# Autodesk Inventor assembly: Joint_0_1
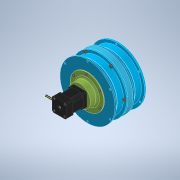
[picture p0: Inventor's stored thumbnail of the model, 180x180]
Saved by Autodesk Inventor 2021 (Build 250183000, 183)
## iProperties
Created: 2020-05-11
Part Number: Joint_0_1
Document SubType Name: Assembly
Designer: avi41
Mass: 3564.7 g
Surface Area: 4281.87 cm^2
Volume: 931.801 cm^3
Density: 3.8256 g/cm^3
Author: avi41
## Documents named in this file (15)
- C:\Users\avi41\Desktop\Robot Arm\CAD_files\Joint_0_1.iam
- C:\Users\avi41\Desktop\Robot Arm\CAD_files\DB41M024030-A.ipt
- C:\Users\avi41\Desktop\Robot Arm\CAD_files\PlanetaryGearbox_stage.iam
- C:\Users\avi41\Desktop\Robot Arm\CAD_files\Adapter_stages_planetary.ipt
- C:\Users\avi41\Documents\Inventor\Content Center Files\R2020\en-US\ANSI B18.3.4M(2)\ANSI B18.3.4M - M4 x 0.7 x 30(1).ipt
- C:\Users\avi41\Documents\Inventor\Content Center Files\R2020\en-US\ISO 4032(1)\ISO 4032 - M4DIN EN.ipt
- C:\Users\avi41\Desktop\Robot Arm\CAD_files\Adapter_motor_planetarygearbox.ipt
- C:\Users\avi41\Documents\Inventor\Content Center Files\R2020\en-US\ANSI B18.3.4M(2)\ANSI B18.3.4M - M3 x 0.5 x 8(1).ipt
- C:\Users\avi41\Documents\Inventor\Content Center Files\R2020\en-US\ISO 8738(1)\ISO 8738 - 3(1).ipt
- C:\Users\avi41\Documents\Inventor\Content Center Files\R2020\en-US\ISO 8738(1)\ISO 8738 - 4(1).ipt
- C:\Users\avi41\Desktop\Robot Arm\CAD_files\MB029-F_1.ipt
- C:\Users\avi41\Desktop\Robot Arm\CAD_files\MRA029BC010DSE00.iam
- C:\Users\avi41\Documents\Inventor\Content Center Files\R2021\en-US\ISO 7046-1 Z(2)\ISO 7046-1 - M2 x 12 - 4.8 - ZNF EN ISO.ipt
- C:\Users\avi41\Documents\Inventor\Content Center Files\R2021\en-US\ISO 4032(1)\ISO 4032 - M2DIN EN.ipt
- C:\Users\avi41\Documents\Inventor\Content Center Files\R2021\en-US\ISO 7046-1 Z(2)\ISO 7046-1 - M3 x 10 - 4.8 - ZNF EN ISO.ipt
## Components (55 placed, 14 different names)
1. PlanetaryGearbox_stage:1 [sub-assembly] — Mate:1, Mate:2, Flush:1, Mate:3, Mate:5, Mate:6, Mate:7, Mate:9, Mate:10, Mate:11, Mate:12, Mate:13, Mate:14, Mate:38, Mate:39, Mate:40, Mate:42, Mate:43, Mate:44, Mate:53, Mate:54, Mate:55, Mate:56
2. DB41M024030-A:1 — Mate:3, Mate:15, Mate:16, Mate:29
3. PlanetaryGearbox_stage:2 [sub-assembly] — Mate:5, Mate:6, Mate:8, Mate:11
4. Adapter_stages_planetary:1 — Mate:7, Mate:8, Mate:9, Mate:10
5. Adapter_motor_planetarygearbox:1 — Mate:12, Mate:13, Mate:14, Mate:15, Mate:16, Mate:29, Mate:58, Mate:59, Mate:60, Mate:61, Flush:2, Flush:3, Flush:4, Flush:5, Mate:62, Mate:63, Mate:64
6. MB029-F_1:1 — Mate:62, Mate:63, Mate:64
7. MRA029BC010DSE00:1 [sub-assembly] — Mate:38, Mate:39, Mate:40, Mate:41, Mate:45, Mate:46, Mate:47, Mate:48
8. DIN EN 24032 M2:1 — Mate:50, Mate:55
9. DIN EN 24032 M2:2 — Mate:49, Mate:56
10. DIN EN 24032 M2:3 — Mate:52, Mate:54
11. DIN EN 24032 M2:4 — Mate:51, Mate:53
12. NF EN ISO 7046-1 - Z M2 x 12 - 4.8 - Z:1 — Mate:43, Mate:46, Mate:50
13. NF EN ISO 7046-1 - Z M2 x 12 - 4.8 - Z:2 — Mate:42, Mate:45, Mate:49
14. NF EN ISO 7046-1 - Z M2 x 12 - 4.8 - Z:3 — Mate:44, Mate:47, Mate:51
15. NF EN ISO 7046-1 - Z M2 x 12 - 4.8 - Z:4 — Mate:41, Mate:48, Mate:52
16. DIN EN 28738 3:5
17. DIN EN 28738 3:6
18. DIN EN 28738 3:7
19. DIN EN 28738 3:8
20. DIN EN 28738 3:9
21. DIN EN 28738 3:10
22. NF EN ISO 7046-1 - Z M3 x 10 - 4.8 - Z:3 — Mate:60, Flush:2
23. Forged Hexagon Socket Button Head Cap Screw - Metric M3 x 0.5 x 8:2
24. NF EN ISO 7046-1 - Z M3 x 10 - 4.8 - Z:4 — Mate:59, Flush:4
25. Forged Hexagon Socket Button Head Cap Screw - Metric M3 x 0.5 x 8:4
26. Forged Hexagon Socket Button Head Cap Screw - Metric M3 x 0.5 x 8:5
27. NF EN ISO 7046-1 - Z M3 x 10 - 4.8 - Z:2 — Mate:58, Flush:5
28. Forged Hexagon Socket Button Head Cap Screw - Metric M3 x 0.5 x 8:7
29. Forged Hexagon Socket Button Head Cap Screw - Metric M3 x 0.5 x 8:8
30. NF EN ISO 7046-1 - Z M3 x 10 - 4.8 - Z:1 — Mate:61, Flush:3
31. Forged Hexagon Socket Button Head Cap Screw - Metric M3 x 0.5 x 8:10
32. DIN EN 28738 4:1
33. DIN EN 28738 4:2
34. DIN EN 28738 4:3
35. DIN EN 28738 4:4
36. DIN EN 28738 4:5
37. DIN EN 28738 4:6
38. DIN EN 28738 4:7
39. DIN EN 28738 4:8
40. DIN EN 28738 4:9
41. DIN EN 28738 4:10
42. DIN EN 28738 4:11
43. DIN EN 28738 4:12
44. Forged Hexagon Socket Button Head Cap Screw - Metric M4 x 0.7 x 30:1
45. Forged Hexagon Socket Button Head Cap Screw - Metric M4 x 0.7 x 30:2
46. Forged Hexagon Socket Button Head Cap Screw - Metric M4 x 0.7 x 30:3
47. Forged Hexagon Socket Button Head Cap Screw - Metric M4 x 0.7 x 30:4
48. Forged Hexagon Socket Button Head Cap Screw - Metric M4 x 0.7 x 30:5
49. Forged Hexagon Socket Button Head Cap Screw - Metric M4 x 0.7 x 30:6
50. DIN EN 24032 M4:1
51. DIN EN 24032 M4:2
52. DIN EN 24032 M4:3
53. DIN EN 24032 M4:4
54. DIN EN 24032 M4:5
55. DIN EN 24032 M4:6
## Relationships (89: Mate 54, Insert 30, Flush 5)
- Mate:1: PlanetaryGearbox_stage:1
- Mate:2: PlanetaryGearbox_stage:1
- Flush:1: PlanetaryGearbox_stage:1
- Mate:3: PlanetaryGearbox_stage:1 ↔ DB41M024030-A:1
- Mate:5: PlanetaryGearbox_stage:1 ↔ PlanetaryGearbox_stage:2
- Mate:6: PlanetaryGearbox_stage:1 ↔ PlanetaryGearbox_stage:2
- Mate:7: PlanetaryGearbox_stage:1 ↔ Adapter_stages_planetary:1
- Mate:8: PlanetaryGearbox_stage:2 ↔ Adapter_stages_planetary:1
- Mate:9: PlanetaryGearbox_stage:1 ↔ Adapter_stages_planetary:1
- [Insert]: PlanetaryGearbox_stage:2 ↔ DIN EN 28738 4:1
- [Insert]: PlanetaryGearbox_stage:2 ↔ DIN EN 28738 4:2
- [Insert]: PlanetaryGearbox_stage:2 ↔ DIN EN 28738 4:3
- [Insert]: PlanetaryGearbox_stage:2 ↔ DIN EN 28738 4:4
- [Insert]: PlanetaryGearbox_stage:2 ↔ DIN EN 28738 4:5
- [Insert]: PlanetaryGearbox_stage:2 ↔ DIN EN 28738 4:6
- [Insert]: PlanetaryGearbox_stage:1 ↔ DIN EN 28738 4:7
- [Insert]: PlanetaryGearbox_stage:1 ↔ DIN EN 28738 4:8
- [Insert]: PlanetaryGearbox_stage:1 ↔ DIN EN 28738 4:9
- [Insert]: PlanetaryGearbox_stage:1 ↔ DIN EN 28738 4:10
- [Insert]: PlanetaryGearbox_stage:1 ↔ DIN EN 28738 4:11
- [Insert]: PlanetaryGearbox_stage:1 ↔ DIN EN 28738 4:12
- Mate:10: PlanetaryGearbox_stage:1 ↔ Adapter_stages_planetary:1
- Mate:11: PlanetaryGearbox_stage:1 ↔ PlanetaryGearbox_stage:2
- [Insert]: DIN EN 28738 4:3 ↔ Forged Hexagon Socket Button Head Cap Screw - Metric M4 x 0.7 x 30:1
- [Insert]: DIN EN 28738 4:2 ↔ Forged Hexagon Socket Button Head Cap Screw - Metric M4 x 0.7 x 30:2
- [Insert]: DIN EN 28738 4:1 ↔ Forged Hexagon Socket Button Head Cap Screw - Metric M4 x 0.7 x 30:3
- [Insert]: DIN EN 28738 4:6 ↔ Forged Hexagon Socket Button Head Cap Screw - Metric M4 x 0.7 x 30:4
- [Insert]: DIN EN 28738 4:5 ↔ Forged Hexagon Socket Button Head Cap Screw - Metric M4 x 0.7 x 30:5
- [Insert]: DIN EN 28738 4:4 ↔ Forged Hexagon Socket Button Head Cap Screw - Metric M4 x 0.7 x 30:6
- [Insert]: DIN EN 28738 4:11 ↔ DIN EN 24032 M4:1
- [Insert]: DIN EN 28738 4:10 ↔ DIN EN 24032 M4:2
- [Insert]: DIN EN 28738 4:9 ↔ DIN EN 24032 M4:3
- [Insert]: DIN EN 28738 4:8 ↔ DIN EN 24032 M4:4
- [Insert]: DIN EN 28738 4:7 ↔ DIN EN 24032 M4:5
- [Insert]: DIN EN 28738 4:12 ↔ DIN EN 24032 M4:6
- Mate:12: PlanetaryGearbox_stage:1 ↔ Adapter_motor_planetarygearbox:1
- Mate:13: PlanetaryGearbox_stage:1 ↔ Adapter_motor_planetarygearbox:1
- Mate:14: PlanetaryGearbox_stage:1 ↔ Adapter_motor_planetarygearbox:1
- Mate:15: DB41M024030-A:1 ↔ Adapter_motor_planetarygearbox:1
- Mate:16: DB41M024030-A:1 ↔ Adapter_motor_planetarygearbox:1
- [Insert]: Adapter_motor_planetarygearbox:1 ↔ DIN EN 28738 3:5
- [Insert]: Adapter_motor_planetarygearbox:1 ↔ DIN EN 28738 3:6
- [Insert]: Adapter_motor_planetarygearbox:1 ↔ DIN EN 28738 3:7
- [Insert]: Adapter_motor_planetarygearbox:1 ↔ DIN EN 28738 3:8
- [Insert]: Adapter_motor_planetarygearbox:1 ↔ DIN EN 28738 3:9
- [Insert]: Adapter_motor_planetarygearbox:1 ↔ DIN EN 28738 3:10
- [Mate]: DIN EN 28738 3:9 ↔ Forged Hexagon Socket Button Head Cap Screw - Metric M3 x 0.5 x 8:10
- [Mate]: DIN EN 28738 3:9 ↔ Forged Hexagon Socket Button Head Cap Screw - Metric M3 x 0.5 x 8:10
- [Mate]: DIN EN 28738 3:6 ↔ Forged Hexagon Socket Button Head Cap Screw - Metric M3 x 0.5 x 8:2
- [Mate]: DIN EN 28738 3:6 ↔ Forged Hexagon Socket Button Head Cap Screw - Metric M3 x 0.5 x 8:2
- [Mate]: DIN EN 28738 3:5 ↔ Forged Hexagon Socket Button Head Cap Screw - Metric M3 x 0.5 x 8:4
- [Mate]: DIN EN 28738 3:5 ↔ Forged Hexagon Socket Button Head Cap Screw - Metric M3 x 0.5 x 8:4
- [Mate]: DIN EN 28738 3:8 ↔ Forged Hexagon Socket Button Head Cap Screw - Metric M3 x 0.5 x 8:8
- [Mate]: DIN EN 28738 3:8 ↔ Forged Hexagon Socket Button Head Cap Screw - Metric M3 x 0.5 x 8:8
- [Mate]: DIN EN 28738 3:7 ↔ Forged Hexagon Socket Button Head Cap Screw - Metric M3 x 0.5 x 8:7
- [Mate]: DIN EN 28738 3:7 ↔ Forged Hexagon Socket Button Head Cap Screw - Metric M3 x 0.5 x 8:7
- [Mate]: DIN EN 28738 3:10 ↔ Forged Hexagon Socket Button Head Cap Screw - Metric M3 x 0.5 x 8:5
- [Mate]: DIN EN 28738 3:10 ↔ Forged Hexagon Socket Button Head Cap Screw - Metric M3 x 0.5 x 8:5
- Mate:29: DB41M024030-A:1 ↔ Adapter_motor_planetarygearbox:1
- Mate:38: PlanetaryGearbox_stage:1 ↔ MRA029BC010DSE00:1
- Mate:39: PlanetaryGearbox_stage:1 ↔ MRA029BC010DSE00:1
- Mate:40: PlanetaryGearbox_stage:1 ↔ MRA029BC010DSE00:1
- Mate:41: MRA029BC010DSE00:1 ↔ NF EN ISO 7046-1 - Z M2 x 12 - 4.8 - Z:4
- Mate:42: PlanetaryGearbox_stage:1 ↔ NF EN ISO 7046-1 - Z M2 x 12 - 4.8 - Z:2
- Mate:43: PlanetaryGearbox_stage:1 ↔ NF EN ISO 7046-1 - Z M2 x 12 - 4.8 - Z:1
- Mate:44: PlanetaryGearbox_stage:1 ↔ NF EN ISO 7046-1 - Z M2 x 12 - 4.8 - Z:3
- Mate:45: MRA029BC010DSE00:1 ↔ NF EN ISO 7046-1 - Z M2 x 12 - 4.8 - Z:2
- Mate:46: MRA029BC010DSE00:1 ↔ NF EN ISO 7046-1 - Z M2 x 12 - 4.8 - Z:1
- Mate:47: MRA029BC010DSE00:1 ↔ NF EN ISO 7046-1 - Z M2 x 12 - 4.8 - Z:3
- Mate:48: MRA029BC010DSE00:1 ↔ NF EN ISO 7046-1 - Z M2 x 12 - 4.8 - Z:4
- Mate:49: DIN EN 24032 M2:2 ↔ NF EN ISO 7046-1 - Z M2 x 12 - 4.8 - Z:2
- Mate:50: DIN EN 24032 M2:1 ↔ NF EN ISO 7046-1 - Z M2 x 12 - 4.8 - Z:1
- Mate:51: DIN EN 24032 M2:4 ↔ NF EN ISO 7046-1 - Z M2 x 12 - 4.8 - Z:3
- Mate:52: DIN EN 24032 M2:3 ↔ NF EN ISO 7046-1 - Z M2 x 12 - 4.8 - Z:4
- Mate:53: PlanetaryGearbox_stage:1 ↔ DIN EN 24032 M2:4
- Mate:54: PlanetaryGearbox_stage:1 ↔ DIN EN 24032 M2:3
- Mate:55: PlanetaryGearbox_stage:1 ↔ DIN EN 24032 M2:1
- Mate:56: PlanetaryGearbox_stage:1 ↔ DIN EN 24032 M2:2
- Mate:58: Adapter_motor_planetarygearbox:1 ↔ NF EN ISO 7046-1 - Z M3 x 10 - 4.8 - Z:2
- Mate:59: Adapter_motor_planetarygearbox:1 ↔ NF EN ISO 7046-1 - Z M3 x 10 - 4.8 - Z:4
- Mate:60: Adapter_motor_planetarygearbox:1 ↔ NF EN ISO 7046-1 - Z M3 x 10 - 4.8 - Z:3
- Mate:61: Adapter_motor_planetarygearbox:1 ↔ NF EN ISO 7046-1 - Z M3 x 10 - 4.8 - Z:1
- Flush:2: Adapter_motor_planetarygearbox:1 ↔ NF EN ISO 7046-1 - Z M3 x 10 - 4.8 - Z:3
- Flush:3: Adapter_motor_planetarygearbox:1 ↔ NF EN ISO 7046-1 - Z M3 x 10 - 4.8 - Z:1
- Flush:4: Adapter_motor_planetarygearbox:1 ↔ NF EN ISO 7046-1 - Z M3 x 10 - 4.8 - Z:4
- Flush:5: Adapter_motor_planetarygearbox:1 ↔ NF EN ISO 7046-1 - Z M3 x 10 - 4.8 - Z:2
- Mate:62: Adapter_motor_planetarygearbox:1 ↔ MB029-F_1:1
- Mate:63: Adapter_motor_planetarygearbox:1 ↔ MB029-F_1:1
- Mate:64: Adapter_motor_planetarygearbox:1 ↔ MB029-F_1:1
